# Autodesk Inventor assembly: test
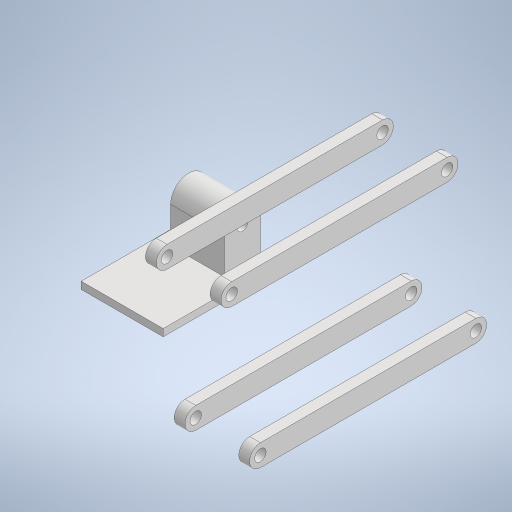
[picture p0: Inventor's stored thumbnail of the model, 512x512]
Saved by Autodesk Inventor 2023 (Build 270158000, 158)
## iProperties
Created: 2024-05-12
Part Number: test
Document SubType Name: Assembly
Designer: kamil
Author: kamil
## Documents named in this file (3)
- C:\Users\kamil\Documents\PROJECTS - repos\ModBot---Projekt-Zespolowy\mechanics\modul_chwytaka\test.iam
- C:\Users\kamil\Documents\PROJECTS - repos\ModBot---Projekt-Zespolowy\mechanics\belka.ipt
- C:\Users\kamil\Documents\PROJECTS - repos\ModBot---Projekt-Zespolowy\mechanics\modul_chwytaka\uchwyt.ipt
## Components (5 placed, 2 different names)
1. belka:1 — Zestawiające:3, Zestawiające:4, Zestawiające:5, Równoległe:1
2. belka:2 — Zestawiające:3, Zestawiające:4, Zestawiające:5
3. belka:3 — Zestawiające:1, Zestawiające:2, Zestawiające:6, Równoległe:1
4. belka:4 — Zestawiające:1, Zestawiające:2, Zestawiające:6
5. uchwyt:1
## Relationships (7: Mate 6, Flush 1)
- Zestawiające:1 [Mate]: belka:3 ↔ belka:4
- Zestawiające:2 [Mate]: belka:3 ↔ belka:4
- Zestawiające:3 [Mate]: belka:1 ↔ belka:2
- Zestawiające:4 [Mate]: belka:1 ↔ belka:2
- Zestawiające:5 [Mate] (15 mm): belka:1 ↔ belka:2
- Zestawiające:6 [Mate] (15 mm): belka:3 ↔ belka:4
- Równoległe:1 [Flush]: belka:1 ↔ belka:3
